# Autodesk Inventor assembly: LegAssembly
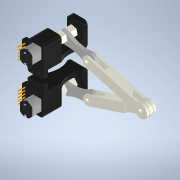
[picture p0: Inventor's stored thumbnail of the model, 180x180]
Saved by Autodesk Inventor 2022 (Build 260153000, 153)
## iProperties
Created: 2021-12-08
Part Number: LegAssembly
Document SubType Name: Assembly
Designer: JK
Author: JK
## Documents named in this file (7)
- C:\Users\JK\Documents\Inventor\N20 Leg Actuator\N20-Leg-Actuator\CADfiles\N20Module\LegAssembly.iam
- C:\Users\JK\Documents\Inventor\N20 Leg Actuator\N20-Leg-Actuator\CADfiles\N20Module\N20Module.iam
- C:\Users\JK\Documents\Inventor\N20 Leg Actuator\N20-Leg-Actuator\CADfiles\N20Module\ShortLink.ipt
- C:\Users\JK\Documents\Inventor\N20 Leg Actuator\N20-Leg-Actuator\CADfiles\N20Module\683zz.ipt
- C:\Users\JK\Documents\Inventor\N20 Leg Actuator\N20-Leg-Actuator\CADfiles\N20Module\LinkC SB.ipt
- C:\Users\JK\Documents\Inventor\N20 Leg Actuator\N20-Leg-Actuator\CADfiles\N20Module\LinkB SB.ipt
- C:\Users\JK\Documents\Inventor\N20 Leg Actuator\N20-Leg-Actuator\CADfiles\N20Module\N20Module_MIR.iam
## Components (9 placed, 6 different names)
1. N20Module:1 [sub-assembly] — Coincidencia:1, Coincidencia:2, Coincidencia:3, Nivelación:6, Nivelación:7, Coincidencia:19
2. ShortLink:1 — Coincidencia:1, Coincidencia:2, Coincidencia:3, Coincidencia:4, Nivelación:1
3. 683zz:1 — Coincidencia:4, Nivelación:1, Coincidencia:10, Coincidencia:11
4. 683zz:2 — Coincidencia:9, Coincidencia:13, Coincidencia:14, Nivelación:5
5. ShortLink:2 — Coincidencia:9, Nivelación:5, Coincidencia:20, Coincidencia:22
6. LinkC SB:1 — Coincidencia:10, Coincidencia:11, Coincidencia:12, Nivelación:4
7. 683zz:3 — Coincidencia:12, Nivelación:4, Coincidencia:15, Coincidencia:21
8. LinkB SB:1 — Coincidencia:13, Coincidencia:14, Coincidencia:15, Coincidencia:21
9. N20Module_MIR:1 [sub-assembly] — Nivelación:6, Nivelación:7, Coincidencia:19, Coincidencia:20, Coincidencia:22
## Relationships (20: Mate 15, Flush 5)
- Coincidencia:1 [Mate] (0.1 mm): N20Module:1 ↔ ShortLink:1
- Coincidencia:2 [Mate] (0.1 mm): N20Module:1 ↔ ShortLink:1
- Coincidencia:3 [Mate] (0.1 mm): N20Module:1 ↔ ShortLink:1
- Coincidencia:4 [Mate]: ShortLink:1 ↔ 683zz:1
- Nivelación:1 [Flush]: ShortLink:1 ↔ 683zz:1
- Coincidencia:9 [Mate]: 683zz:2 ↔ ShortLink:2
- Coincidencia:10 [Mate]: 683zz:1 ↔ LinkC SB:1
- Coincidencia:11 [Mate] (0.1 mm): 683zz:1 ↔ LinkC SB:1
- Coincidencia:12 [Mate]: LinkC SB:1 ↔ 683zz:3
- Nivelación:4 [Flush]: LinkC SB:1 ↔ 683zz:3
- Coincidencia:13 [Mate]: 683zz:2 ↔ LinkB SB:1
- Coincidencia:14 [Mate] (0.1 mm): 683zz:2 ↔ LinkB SB:1
- Nivelación:5 [Flush]: 683zz:2 ↔ ShortLink:2
- Coincidencia:15 [Mate]: 683zz:3 ↔ LinkB SB:1
- Nivelación:6 [Flush]: N20Module:1 ↔ N20Module_MIR:1
- Nivelación:7 [Flush]: N20Module:1 ↔ N20Module_MIR:1
- Coincidencia:19 [Mate] (3.7 mm): N20Module:1 ↔ N20Module_MIR:1
- Coincidencia:20 [Mate] (0.1 mm): ShortLink:2 ↔ N20Module_MIR:1
- Coincidencia:21 [Mate]: 683zz:3 ↔ LinkB SB:1
- Coincidencia:22 [Mate] (0.1 mm): ShortLink:2 ↔ N20Module_MIR:1
